# Autodesk Inventor assembly: Rover
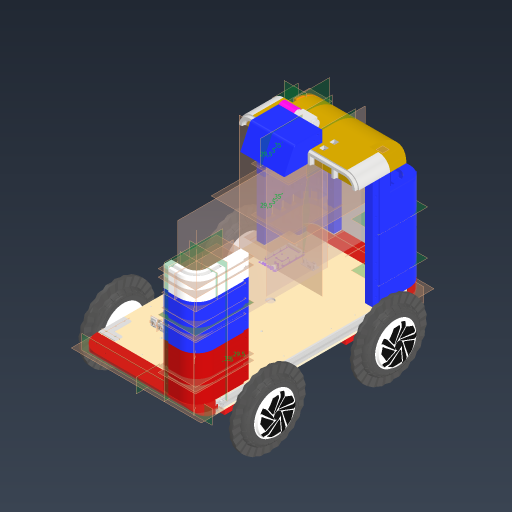
[picture p0: Inventor's stored thumbnail of the model, 512x512]
Saved by Autodesk Inventor 2023.2 (Build 272271030, 271C)
## iProperties
Created: 2024-10-30
Part Number: Rover
Document SubType Name: Assembly
Designer: I9232
Author: I9232
## Documents named in this file (34)
- D:\!Rover\Rover\Rover_construction\Rover.iam
- D:\!Rover\Rover\Rover_construction\platform.ipt
- D:\!Rover\Rover\Rover_construction\Motor, BLDC, Hoverboard Wheel, 8.0in.ipt
- D:\!Rover\Rover\Rover_construction\Profil 20x20.ipt
- D:\!Rover\Rover\Rover_construction\Крепление мотора.iam
- D:\!Rover\Rover\Rover_construction\Уголок для профиля.ipt
- D:\!Rover\Rover\Rover_construction\Профиль 30x30\Профиль 30x30.ipt
- D:\!Rover\Rover\Rover_construction\Т-образный соединитель\Т-образный соединитель.ipt
- D:\!Rover\Rover\Rover_construction\Подъёмник.iam
- D:\!Rover\Rover\Rover_construction\Боковая часть корпуса.ipt
- D:\!Rover\Rover\Rover_construction\Передняя_Задняя фанера.ipt
- D:\!Rover\Rover\Rover_construction\Сборка_столбик_зад.iam
- D:\!Rover\Rover\Rover_construction\Столбик.ipt
- D:\!Rover\Rover\Rover_construction\Крышка.ipt
- D:\!Rover\Rover\Rover_construction\Уголок крышки.ipt
- D:\!Rover\Rover\Rover_construction\Крышка.iam
- D:\!Rover\Rover\Rover_construction\Вторая часть петли.ipt
- D:\!Rover\Rover\Rover_construction\рдс150.ipt
- D:\!Rover\Rover\Rover_construction\Ушко петли крышки2,0.ipt
- D:\!Rover\Rover\Rover_construction\Arduino_Due\Arduino_Due.ipt
- D:\!Rover\Rover\Rover_construction\LM2596 DC-DC stepdown voltage converter\LM2596 DC-DC stepdown voltage converter.ipt
- D:\!Rover\Rover\Rover_construction\DS51_Arm_Disc\DS51_Arm_Disc.ipt
- D:\!Rover\Rover\Rover_construction\Крепление датчика ульразвука.iam
- D:\!Rover\Rover\Rover_construction\Нижний край корпуса.ipt
- D:\!Rover\Rover\Rover_construction\Задний_столб.iam
- D:\!Rover\Rover\Rover_construction\Столб_переда_корпуса_2.0.iam
- D:\!Rover\Rover\Rover_construction\Столб_переда_корпуса_2.0_MIR.iam
- D:\!Rover\Rover\Rover_construction\Уголок_передней_крышки_2.0.ipt
- D:\!Rover\Rover\Rover_construction\Уголок_передней_крышки_2.0_MIR.ipt
- D:\!Rover\Rover\Rover_construction\Проставка_платформы_и_столба.ipt
- D:\!Rover\Rover\Rover_construction\Сборка_крепления_камеры.iam
- D:\!Rover\Rover\Rover_construction\Передняя_фанера.ipt
- D:\!Rover\Rover\Rover_construction\Козырёк_для_камеры.ipt
- D:\!Rover\Rover\Rover_construction\Козырёк_версия_2.ipt
## Components (56 placed, 33 different names)
1. platform:1 — Совмещение:1, Совмещение:2, Совмещение:169, Заподлицо:1, Заподлицо:2, Совмещение:170, Совмещение:171, Совмещение:172, Заподлицо:3, Заподлицо:4, Заподлицо:5, Заподлицо:6, Совмещение:180, Заподлицо:11, Совмещение:189, Заподлицо:24, Заподлицо:25, Совмещение:190, Заподлицо:26, Заподлицо:27, Заподлицо:28, Совмещение:191, Заподлицо:29, Совмещение:192, Заподлицо:30, Заподлицо:31, Заподлицо:37, Заподлицо:63
2. Т-образный соединитель:1 — Заподлицо:21, Совмещение:188
3. Т-образный соединитель:2 — Совмещение:187, Заподлицо:23
4. Подъёмник:1 [sub-assembly] — Совмещение:355, Совмещение:356, Совмещение:357
5. platform:2 — Заподлицо:37, Заподлицо:38, Совмещение:313, Совмещение:314, Совмещение:315, Совмещение:316, Совмещение:317, Заподлицо:39, Заподлицо:40, Заподлицо:41, Заподлицо:42, Заподлицо:43, Заподлицо:44, Заподлицо:46, Заподлицо:47, Совмещение:350, Совмещение:351, Совмещение:355, Заподлицо:58, Заподлицо:62, Заподлицо:64, Заподлицо:68
6. Боковая часть корпуса:1 — Совмещение:327, Совмещение:328, Заподлицо:45, Симметрия:4
7. Боковая часть корпуса:2 — Совмещение:321, Совмещение:322, Совмещение:323, Симметрия:4
8. Передняя_Задняя фанера:2 — Совмещение:324, Совмещение:325, Совмещение:326, Совмещение:368, Совмещение:369, Совмещение:370
9. Передняя_Задняя фанера:4 — Совмещение:330, Совмещение:331, Заподлицо:48
10. Сборка_столбик_зад:1 [sub-assembly] — Совмещение:318, Заподлицо:39, Заподлицо:40, Совмещение:322, Совмещение:323, Совмещение:324, Совмещение:325, Совмещение:357
11. Сборка_столбик_зад:2 [sub-assembly] — Совмещение:319, Заподлицо:41, Заподлицо:42, Совмещение:326, Совмещение:327, Совмещение:328, Заподлицо:45
12. Столбик:1 — Совмещение:320, Заподлицо:43, Заподлицо:44, Совмещение:321, Совмещение:331, Совмещение:352, Совмещение:353
13. Столбик:2 — Совмещение:329, Заподлицо:46, Заподлицо:47, Совмещение:330, Заподлицо:48
14. Крышка:1 — Совмещение:383, Совмещение:388, Совмещение:389, Совмещение:393, Заподлицо:67, Совмещение:399, Совмещение:400, Совмещение:405, Совмещение:407, Совмещение:408, Совмещение:412
15. Уголок крышки:2 — Совмещение:392, Заподлицо:66, Совмещение:393
16. Крышка:2 [sub-assembly] — Совмещение:396, Совмещение:398
17. Вторая часть петли:2 — Совмещение:347, Заподлицо:54, Совмещение:348, Заподлицо:67, Совмещение:398
18. рдс150:1 — Совмещение:347, Заподлицо:54, Совмещение:348, Совмещение:358, Совмещение:359, Совмещение:360, Совмещение:361
19. Ушко петли крышки2,0:1 — Совмещение:362, Совмещение:363, Совмещение:364
20. Arduino_Due:1 — Совмещение:350, Совмещение:352, Совмещение:353, Совмещение:354
21. LM2596 DC-DC stepdown voltage converter:1 — Совмещение:351, Совмещение:354
22. DS51_Arm_Disc:1 — Совмещение:359, Совмещение:361, Совмещение:362, Совмещение:363, Совмещение:364
23. DS51_Arm_Disc:2 — Совмещение:358, Совмещение:360
24. Крепление датчика ульразвука:1 [sub-assembly] — Совмещение:368, Совмещение:369, Совмещение:370
25. Нижний край корпуса:1 — Совмещение:376, Заподлицо:58, Заподлицо:59, Заподлицо:60, Совмещение:382
26. Нижний край корпуса:2 — Заподлицо:60, Совмещение:377, Заподлицо:61, Совмещение:379, Совмещение:385, Совмещение:402, Совмещение:403
27. Задний_столб:1 [sub-assembly] — Совмещение:381, Заподлицо:63, Совмещение:382, Совмещение:396
28. Столб_переда_корпуса_2.0:1 [sub-assembly] — Заподлицо:62, Совмещение:379, Совмещение:380, Совмещение:383, Совмещение:388, Совмещение:389, Совмещение:392, Заподлицо:66, Совмещение:401, Совмещение:411
29. Столб_переда_корпуса_2.0_MIR:1 [sub-assembly] — Совмещение:384, Совмещение:385, Заподлицо:64, Совмещение:404, Совмещение:410
30. Уголок_передней_крышки_2.0:1 — Совмещение:399, Совмещение:400, Совмещение:401
31. Уголок_передней_крышки_2.0_MIR:1 — Совмещение:404, Совмещение:405
32. Проставка_платформы_и_столба:1 — Совмещение:402, Заподлицо:68, Совмещение:403
33. Сборка_крепления_камеры:1 [sub-assembly] — Совмещение:407, Совмещение:408, Совмещение:413
34. Передняя_фанера:1 — Совмещение:410, Совмещение:411, Совмещение:412, Совмещение:413, Совмещение:414, Совмещение:415, Совмещение:416, Совмещение:417, Заподлицо:69
35. Козырёк_для_камеры:1 — Совмещение:414, Совмещение:415
36. Козырёк_версия_2:1 — Совмещение:416, Совмещение:417, Заподлицо:69
37. Мотор гироскутера — Совмещение:196, Совмещение:197, Совмещение:198
38. Motor, BLDC, Hoverboard Wheel, 8.0in:4 — Совмещение:199, Совмещение:200, Совмещение:201
39. Motor, BLDC, Hoverboard Wheel, 8.0in:5 — Совмещение:193, Совмещение:194, Совмещение:195
40. Motor, BLDC, Hoverboard Wheel, 8.0in:6 — Совмещение:202, Совмещение:203, Совмещение:204
41. Profil 20x20:1 — Симметрия:3, Заподлицо:14, Совмещение:184, Заподлицо:18
42. Profil 20x20:2 — Симметрия:3, Заподлицо:12, Совмещение:181, Заподлицо:13
43. Profil 20x20:3 — Заподлицо:18
44. Профиль 30x30:5 — Совмещение:179, Совмещение:180, Заподлицо:11, Заподлицо:21, Заподлицо:23
45. Профиль 30x30:2 — Совмещение:171, Совмещение:173, Заподлицо:3, Заподлицо:7, Заподлицо:12, Совмещение:181, Заподлицо:35, Заподлицо:38
46. Профиль 30x30:3 — Совмещение:170, Заподлицо:5, Заподлицо:6, Совмещение:188, Совмещение:313, Совмещение:371, Совмещение:372, Совмещение:377, Заподлицо:61
47. Профиль 30x30:4 — Совмещение:172, Совмещение:174, Заподлицо:4, Совмещение:178, Заподлицо:13, Заподлицо:14, Совмещение:184, Совмещение:219
48. Профиль 30x30:1 — Совмещение:169, Заподлицо:1, Заподлицо:2, Совмещение:173, Совмещение:174, Совмещение:179, Совмещение:187, Заподлицо:55, Заподлицо:56, Совмещение:376, Заподлицо:59
49. Крепление мотора:1 [sub-assembly] — Совмещение:189, Заподлицо:24, Заподлицо:25, Совмещение:199, Совмещение:200, Совмещение:201
50. Крепление мотора:2 [sub-assembly] — Совмещение:190, Заподлицо:26, Заподлицо:27, Совмещение:196, Совмещение:197, Совмещение:198
51. Крепление мотора:3 [sub-assembly] — Заподлицо:28, Совмещение:191, Заподлицо:29, Совмещение:202, Совмещение:203, Совмещение:204
52. Крепление мотора:4 [sub-assembly] — Совмещение:192, Заподлицо:30, Заподлицо:31, Совмещение:193, Совмещение:194, Совмещение:195
53. Уголок для профиля:1 — Совмещение:178, Совмещение:317, Совмещение:319, Заподлицо:55, Совмещение:381
54. Уголок для профиля:2 — Заподлицо:7, Совмещение:314, Совмещение:320, Совмещение:371, Совмещение:380
55. Уголок для профиля:3 — Заподлицо:35, Совмещение:316, Совмещение:318, Заподлицо:56
56. Уголок для профиля:4 — Совмещение:219, Совмещение:315, Совмещение:329, Совмещение:372, Совмещение:384
## Relationships (156: Mate 105, Flush 49, Symmetry 2)
- Совмещение:1 [Mate]: platform:1
- Совмещение:2 [Mate]: platform:1
- Симметрия:3 [Symmetry]: Profil 20x20:1 ↔ Profil 20x20:2
- Совмещение:169 [Mate]: platform:1 ↔ Профиль 30x30:1
- Заподлицо:1 [Flush]: platform:1 ↔ Профиль 30x30:1
- Заподлицо:2 [Flush]: platform:1 ↔ Профиль 30x30:1
- Совмещение:170 [Mate]: platform:1 ↔ Профиль 30x30:3
- Совмещение:171 [Mate]: platform:1 ↔ Профиль 30x30:2
- Совмещение:172 [Mate]: platform:1 ↔ Профиль 30x30:4
- Совмещение:173 [Mate]: Профиль 30x30:2 ↔ Профиль 30x30:1
- Заподлицо:3 [Flush]: platform:1 ↔ Профиль 30x30:2
- Совмещение:174 [Mate]: Профиль 30x30:4 ↔ Профиль 30x30:1
- Заподлицо:4 [Flush]: platform:1 ↔ Профиль 30x30:4
- Заподлицо:5 [Flush]: platform:1 ↔ Профиль 30x30:3
- Заподлицо:6 [Flush]: platform:1 ↔ Профиль 30x30:3
- Заподлицо:7 [Flush]: Профиль 30x30:2 ↔ Уголок для профиля:2
- Совмещение:178 [Mate]: Профиль 30x30:4 ↔ Уголок для профиля:1
- Совмещение:179 [Mate]: Профиль 30x30:5 ↔ Профиль 30x30:1
- Совмещение:180 [Mate]: platform:1 ↔ Профиль 30x30:5
- Заподлицо:11 [Flush]: platform:1 ↔ Профиль 30x30:5
- Заподлицо:12 [Flush]: Profil 20x20:2 ↔ Профиль 30x30:2
- Совмещение:181 [Mate]: Profil 20x20:2 ↔ Профиль 30x30:2
- Заподлицо:13 [Flush]: Profil 20x20:2 ↔ Профиль 30x30:4
- Заподлицо:14 [Flush]: Profil 20x20:1 ↔ Профиль 30x30:4
- Совмещение:184 [Mate]: Profil 20x20:1 ↔ Профиль 30x30:4
- Заподлицо:18 [Flush] (-200 mm): Profil 20x20:1 ↔ Profil 20x20:3
- Заподлицо:21 [Flush]: Т-образный соединитель:1 ↔ Профиль 30x30:5
- Совмещение:187 [Mate]: Т-образный соединитель:2 ↔ Профиль 30x30:1
- Заподлицо:23 [Flush]: Т-образный соединитель:2 ↔ Профиль 30x30:5
- Совмещение:188 [Mate]: Т-образный соединитель:1 ↔ Профиль 30x30:3
- Совмещение:189 [Mate]: platform:1 ↔ Крепление мотора:1
- Заподлицо:24 [Flush] (30 mm): platform:1 ↔ Крепление мотора:1
- Заподлицо:25 [Flush]: platform:1 ↔ Крепление мотора:1
- Совмещение:190 [Mate]: platform:1 ↔ Крепление мотора:2
- Заподлицо:26 [Flush] (30 mm): platform:1 ↔ Крепление мотора:2
- Заподлицо:27 [Flush]: platform:1 ↔ Крепление мотора:2
- Заподлицо:28 [Flush] (30 mm): platform:1 ↔ Крепление мотора:3
- Совмещение:191 [Mate]: platform:1 ↔ Крепление мотора:3
- Заподлицо:29 [Flush]: platform:1 ↔ Крепление мотора:3
- Совмещение:192 [Mate]: platform:1 ↔ Крепление мотора:4
- Заподлицо:30 [Flush]: platform:1 ↔ Крепление мотора:4
- Заподлицо:31 [Flush] (30 mm): platform:1 ↔ Крепление мотора:4
- Совмещение:193 [Mate]: Motor, BLDC, Hoverboard Wheel, 8.0in:5 ↔ Крепление мотора:4
- Совмещение:194 [Mate]: Motor, BLDC, Hoverboard Wheel, 8.0in:5 ↔ Крепление мотора:4
- Совмещение:195 [Mate]: Motor, BLDC, Hoverboard Wheel, 8.0in:5 ↔ Крепление мотора:4
- Совмещение:196 [Mate]: Мотор гироскутера ↔ Крепление мотора:2
- Совмещение:197 [Mate]: Мотор гироскутера ↔ Крепление мотора:2
- Совмещение:198 [Mate]: Мотор гироскутера ↔ Крепление мотора:2
- Совмещение:199 [Mate]: Motor, BLDC, Hoverboard Wheel, 8.0in:4 ↔ Крепление мотора:1
- Совмещение:200 [Mate]: Motor, BLDC, Hoverboard Wheel, 8.0in:4 ↔ Крепление мотора:1
- Совмещение:201 [Mate]: Motor, BLDC, Hoverboard Wheel, 8.0in:4 ↔ Крепление мотора:1
- Совмещение:202 [Mate]: Motor, BLDC, Hoverboard Wheel, 8.0in:6 ↔ Крепление мотора:3
- Совмещение:203 [Mate]: Motor, BLDC, Hoverboard Wheel, 8.0in:6 ↔ Крепление мотора:3
- Совмещение:204 [Mate]: Motor, BLDC, Hoverboard Wheel, 8.0in:6 ↔ Крепление мотора:3
- Совмещение:219 [Mate]: Профиль 30x30:4 ↔ Уголок для профиля:4
- Заподлицо:35 [Flush]: Профиль 30x30:2 ↔ Уголок для профиля:3
- Заподлицо:37 [Flush]: platform:1 ↔ platform:2
- Заподлицо:38 [Flush]: platform:2 ↔ Профиль 30x30:2
- Совмещение:313 [Mate]: platform:2 ↔ Профиль 30x30:3
- Совмещение:314 [Mate]: platform:2 ↔ Уголок для профиля:2
- Совмещение:315 [Mate]: platform:2 ↔ Уголок для профиля:4
- Совмещение:316 [Mate]: platform:2 ↔ Уголок для профиля:3
- Совмещение:317 [Mate]: platform:2 ↔ Уголок для профиля:1
- Совмещение:318 [Mate]: Сборка_столбик_зад:1 ↔ Уголок для профиля:3
- Совмещение:319 [Mate]: Сборка_столбик_зад:2 ↔ Уголок для профиля:1
- Заподлицо:39 [Flush]: platform:2 ↔ Сборка_столбик_зад:1
- Заподлицо:40 [Flush]: platform:2 ↔ Сборка_столбик_зад:1
- Заподлицо:41 [Flush]: platform:2 ↔ Сборка_столбик_зад:2
- Заподлицо:42 [Flush]: platform:2 ↔ Сборка_столбик_зад:2
- Совмещение:320 [Mate]: Столбик:1 ↔ Уголок для профиля:2
- Заподлицо:43 [Flush]: platform:2 ↔ Столбик:1
- Заподлицо:44 [Flush]: platform:2 ↔ Столбик:1
- Совмещение:321 [Mate]: Боковая часть корпуса:2 ↔ Столбик:1
- Совмещение:322 [Mate]: Боковая часть корпуса:2 ↔ Сборка_столбик_зад:1
- Совмещение:323 [Mate]: Боковая часть корпуса:2 ↔ Сборка_столбик_зад:1
- Совмещение:324 [Mate]: Передняя_Задняя фанера:2 ↔ Сборка_столбик_зад:1
- Совмещение:325 [Mate]: Передняя_Задняя фанера:2 ↔ Сборка_столбик_зад:1
- Совмещение:326 [Mate]: Передняя_Задняя фанера:2 ↔ Сборка_столбик_зад:2
- Совмещение:327 [Mate]: Боковая часть корпуса:1 ↔ Сборка_столбик_зад:2
- Совмещение:328 [Mate]: Боковая часть корпуса:1 ↔ Сборка_столбик_зад:2
- Заподлицо:45 [Flush]: Боковая часть корпуса:1 ↔ Сборка_столбик_зад:2
- Симметрия:4 [Symmetry]: Боковая часть корпуса:1 ↔ Боковая часть корпуса:2
- Совмещение:329 [Mate]: Столбик:2 ↔ Уголок для профиля:4
- Заподлицо:46 [Flush]: platform:2 ↔ Столбик:2
- Заподлицо:47 [Flush]: platform:2 ↔ Столбик:2
- Совмещение:330 [Mate]: Передняя_Задняя фанера:4 ↔ Столбик:2
- Совмещение:331 [Mate]: Передняя_Задняя фанера:4 ↔ Столбик:1
- Заподлицо:48 [Flush]: Передняя_Задняя фанера:4 ↔ Столбик:2
- Совмещение:347 [Mate]: Вторая часть петли:2 ↔ рдс150:1
- Заподлицо:54 [Flush]: Вторая часть петли:2 ↔ рдс150:1
- Совмещение:348 [Mate]: Вторая часть петли:2 ↔ рдс150:1
- Совмещение:350 [Mate]: platform:2 ↔ Arduino_Due:1
- Совмещение:351 [Mate]: platform:2 ↔ LM2596 DC-DC stepdown voltage converter:1
- Совмещение:352 [Mate] (40 mm): Столбик:1 ↔ Arduino_Due:1
- Совмещение:353 [Mate] (40 mm): Столбик:1 ↔ Arduino_Due:1
- Совмещение:354 [Mate] (20 mm): Arduino_Due:1 ↔ LM2596 DC-DC stepdown voltage converter:1
- Совмещение:355 [Mate]: Подъёмник:1 ↔ platform:2
- Совмещение:356 [Mate]: Подъёмник:1
- Совмещение:357 [Mate] (30 mm): Подъёмник:1 ↔ Сборка_столбик_зад:1
- Совмещение:358 [Mate]: рдс150:1 ↔ DS51_Arm_Disc:2
- Совмещение:359 [Mate]: рдс150:1 ↔ DS51_Arm_Disc:1
- Совмещение:360 [Mate]: рдс150:1 ↔ DS51_Arm_Disc:2
- Совмещение:361 [Mate]: рдс150:1 ↔ DS51_Arm_Disc:1
- Совмещение:362 [Mate]: Ушко петли крышки2,0:1 ↔ DS51_Arm_Disc:1
- Совмещение:363 [Mate] (1 mm): Ушко петли крышки2,0:1 ↔ DS51_Arm_Disc:1
- Совмещение:364 [Mate]: Ушко петли крышки2,0:1 ↔ DS51_Arm_Disc:1
- Совмещение:368 [Mate]: Передняя_Задняя фанера:2 ↔ Крепление датчика ульразвука:1
- Совмещение:369 [Mate]: Передняя_Задняя фанера:2 ↔ Крепление датчика ульразвука:1
- Совмещение:370 [Mate]: Передняя_Задняя фанера:2 ↔ Крепление датчика ульразвука:1
- Совмещение:371 [Mate]: Профиль 30x30:3 ↔ Уголок для профиля:2
- Заподлицо:55 [Flush]: Профиль 30x30:1 ↔ Уголок для профиля:1
- Совмещение:372 [Mate]: Профиль 30x30:3 ↔ Уголок для профиля:4
- Заподлицо:56 [Flush]: Профиль 30x30:1 ↔ Уголок для профиля:3
- Совмещение:376 [Mate]: Нижний край корпуса:1 ↔ Профиль 30x30:1
- Заподлицо:58 [Flush]: platform:2 ↔ Нижний край корпуса:1
- Заподлицо:59 [Flush]: Нижний край корпуса:1 ↔ Профиль 30x30:1
- Заподлицо:60 [Flush]: Нижний край корпуса:1 ↔ Нижний край корпуса:2
- Совмещение:377 [Mate]: Нижний край корпуса:2 ↔ Профиль 30x30:3
- Заподлицо:61 [Flush]: Нижний край корпуса:2 ↔ Профиль 30x30:3
- Заподлицо:62 [Flush]: platform:2 ↔ Столб_переда_корпуса_2.0:1
- Совмещение:379 [Mate]: Нижний край корпуса:2 ↔ Столб_переда_корпуса_2.0:1
- Совмещение:380 [Mate]: Столб_переда_корпуса_2.0:1 ↔ Уголок для профиля:2
- Совмещение:381 [Mate]: Задний_столб:1 ↔ Уголок для профиля:1
- Заподлицо:63 [Flush]: platform:1 ↔ Задний_столб:1
- Совмещение:382 [Mate]: Нижний край корпуса:1 ↔ Задний_столб:1
- Совмещение:383 [Mate]: Крышка:1 ↔ Столб_переда_корпуса_2.0:1
- Совмещение:384 [Mate]: Столб_переда_корпуса_2.0_MIR:1 ↔ Уголок для профиля:4
- Совмещение:385 [Mate]: Нижний край корпуса:2 ↔ Столб_переда_корпуса_2.0_MIR:1
- Заподлицо:64 [Flush]: platform:2 ↔ Столб_переда_корпуса_2.0_MIR:1
- Совмещение:388 [Mate]: Крышка:1 ↔ Столб_переда_корпуса_2.0:1
- Совмещение:389 [Mate]: Крышка:1 ↔ Столб_переда_корпуса_2.0:1
- Совмещение:392 [Mate]: Уголок крышки:2 ↔ Столб_переда_корпуса_2.0:1
- Заподлицо:66 [Flush]: Уголок крышки:2 ↔ Столб_переда_корпуса_2.0:1
- Совмещение:393 [Mate]: Крышка:1 ↔ Уголок крышки:2
- Совмещение:396 [Mate]: Крышка:2 ↔ Задний_столб:1
- Заподлицо:67 [Flush]: Крышка:1 ↔ Вторая часть петли:2
- Совмещение:398 [Mate]: Крышка:2 ↔ Вторая часть петли:2
- Совмещение:399 [Mate]: Крышка:1 ↔ Уголок_передней_крышки_2.0:1
- Совмещение:400 [Mate]: Крышка:1 ↔ Уголок_передней_крышки_2.0:1
- Совмещение:401 [Mate]: Столб_переда_корпуса_2.0:1 ↔ Уголок_передней_крышки_2.0:1
- Совмещение:402 [Mate]: Нижний край корпуса:2 ↔ Проставка_платформы_и_столба:1
- Заподлицо:68 [Flush]: platform:2 ↔ Проставка_платформы_и_столба:1
- Совмещение:403 [Mate]: Нижний край корпуса:2 ↔ Проставка_платформы_и_столба:1
- Совмещение:404 [Mate]: Столб_переда_корпуса_2.0_MIR:1 ↔ Уголок_передней_крышки_2.0_MIR:1
- Совмещение:405 [Mate]: Крышка:1 ↔ Уголок_передней_крышки_2.0_MIR:1
- Совмещение:407 [Mate]: Крышка:1 ↔ Сборка_крепления_камеры:1
- Совмещение:408 [Mate] (4 mm): Крышка:1 ↔ Сборка_крепления_камеры:1
- Совмещение:410 [Mate]: Столб_переда_корпуса_2.0_MIR:1 ↔ Передняя_фанера:1
- Совмещение:411 [Mate]: Столб_переда_корпуса_2.0:1 ↔ Передняя_фанера:1
- Совмещение:412 [Mate]: Крышка:1 ↔ Передняя_фанера:1
- Совмещение:413 [Mate]: Сборка_крепления_камеры:1 ↔ Передняя_фанера:1
- Совмещение:414 [Mate]: Передняя_фанера:1 ↔ Козырёк_для_камеры:1
- Совмещение:415 [Mate]: Передняя_фанера:1 ↔ Козырёк_для_камеры:1
- Совмещение:416 [Mate]: Передняя_фанера:1 ↔ Козырёк_версия_2:1
- Совмещение:417 [Mate]: Передняя_фанера:1 ↔ Козырёк_версия_2:1
- Заподлицо:69 [Flush]: Передняя_фанера:1 ↔ Козырёк_версия_2:1
